# Autodesk Inventor assembly: tether-manipulator-assembly
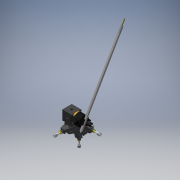
[picture p0: Inventor's stored thumbnail of the model, 180x180]
Saved by Autodesk Inventor 2019 (Build 230136000, 136)
## iProperties
Created: 2019-05-18
Part Number: tether-manipulator-assembly
Document SubType Name: Assembly
Designer: Wilson Lab
Author: Wilson Lab
## Documents named in this file (5)
- C:\code\auditory-behavior-experiments\design-files\tether-assembly\tether-manipulator-assembly.iam
- C:\code\auditory-behavior-experiments\design-files\tether-assembly\tether-assembly.iam
- C:\code\auditory-behavior-experiments\design-files\vr-opto-assembly\T12A2-Solidworks.ipt
- C:\code\auditory-behavior-experiments\design-files\tether-assembly\RM1F-Solidworks.ipt
- C:\code\auditory-behavior-experiments\design-files\vr-opto-assembly\T12XYZ-Solidworks.ipt
## Components (4 placed, 4 different names)
1. tether-assembly:1 [sub-assembly] — Rotational:3
2. T12A2-Solidworks:1 — Rigid:1, Rigid:3
3. RM1F-Solidworks:1 — Rigid:1, Rotational:3
4. T12XYZ-Solidworks:1 — Rigid:3
## Relationships (3: WeldJoint 2, RevoluteJoint 1)
- Rigid:1 [WeldJoint]: T12A2-Solidworks:1 ↔ RM1F-Solidworks:1
- Rotational:3 [RevoluteJoint]: tether-assembly:1 ↔ RM1F-Solidworks:1
- Rigid:3 [WeldJoint]: T12A2-Solidworks:1 ↔ T12XYZ-Solidworks:1
